# Autodesk Inventor assembly: Klappmechanismus Antrieb
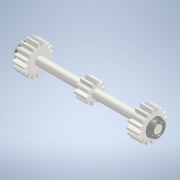
[picture p0: Inventor's stored thumbnail of the model, 180x180]
Saved by Autodesk Inventor 2021 (Build 250183000, 183)
## iProperties
Created: 2021-01-29
Part Number: Klappmechanismus Antrieb
Document SubType Name: Assembly
Designer: Jaro Machnow
Author: Jaro Machnow
## Documents named in this file (5)
- C:\Users\Jaro Machnow\Documents\Vault\Gruppen\Gruppe 2\Entwurf\Amphibienfahrzeug\Wechsel zwischen Land und Wasser\Wechselmechanik\Klappmechanismus Antrieb.iam
- C:\Users\Jaro Machnow\Documents\Vault\Gruppen\Gruppe 2\Entwurfzeichnungen\Jaro Machnow\Klappmechanismus\Welle1.ipt
- C:\Users\Jaro Machnow\Documents\Vault\Gruppen\Gruppe 2\Entwurfzeichnungen\Jaro Machnow\Klappmechanismus\Klappmechanismus Antrieb\Konstruktions-Assistent\Stirnräder2.iam
- C:\Users\Jaro Machnow\Documents\Vault\Gruppen\Gruppe 2\Entwurfzeichnungen\Jaro Machnow\Klappmechanismus\Klappmechanismus Antrieb\Konstruktions-Assistent\Stirnräder3.iam
- C:\Users\Jaro Machnow\Documents\Vault\Gruppen\Gruppe 2\Entwurfzeichnungen\Jaro Machnow\Klappmechanismus\Klappmechanismus Antrieb\Konstruktions-Assistent\Lager1.iam
## Components (6 placed, 3 different names)
1. Welle:1 — Passend:1, Passend:2, Passend:4, Passend:7, Fluchtend:1, Passend:8, Fluchtend:2
2. Stirnräder:1 [sub-assembly] — Passend:1
3. Stirnräder:2 [sub-assembly] — Passend:2
4. Stirnräder:3 [sub-assembly] — Passend:4
5. Lager:2 [sub-assembly] — Passend:7, Fluchtend:1
6. Lager:3 [sub-assembly] — Passend:8, Fluchtend:2
## Relationships (7: Mate 5, Flush 2)
- Passend:1 [Mate]: Welle:1 ↔ Stirnräder:1
- Passend:2 [Mate]: Welle:1 ↔ Stirnräder:2
- Passend:4 [Mate]: Welle:1 ↔ Stirnräder:3
- Passend:7 [Mate]: Welle:1 ↔ Lager:2
- Fluchtend:1 [Flush]: Welle:1 ↔ Lager:2
- Passend:8 [Mate]: Welle:1 ↔ Lager:3
- Fluchtend:2 [Flush]: Welle:1 ↔ Lager:3
